# Autodesk Inventor assembly: Stator
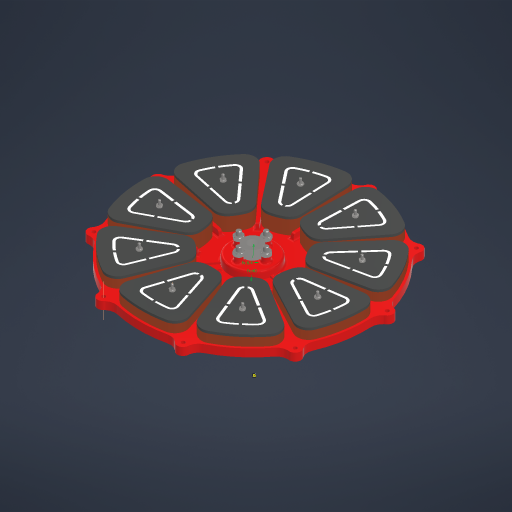
[picture p0: Inventor's stored thumbnail of the model, 512x512]
Saved by Autodesk Inventor 2023.1 (Build 271208000, 208)
## iProperties
Created: 2022-07-30
Part Number: Stator
Document SubType Name: Assembly
Designer: ABL
Author: ABL
## Documents named in this file (11)
- C:\GitHubRepos\PHYS-12-Website\content\portfolio\Final Project\CAD\Axial Flux Motor iProject\Stator.iam
- C:\GitHubRepos\PHYS-12-Website\content\portfolio\Final Project\CAD\Axial Flux Motor iProject\StatorBody.ipt
- C:\GitHubRepos\PHYS-12-Website\content\portfolio\Final Project\CAD\Axial Flux Motor iProject\CoilRing.ipt
- C:\GitHubRepos\PHYS-12-Website\content\portfolio\The Everybolt\MetricSocketBolt.ipt
- C:\GitHubRepos\PHYS-12-Website\content\portfolio\Final Project\CAD\Axial Flux Motor iProject\Fasteners\statorMountBolt.ipt
- C:\GitHubRepos\PHYS-12-Website\content\portfolio\Final Project\CAD\Axial Flux Motor iProject\Fasteners\statorMountHexNut.ipt
- C:\GitHubRepos\PHYS-12-Website\content\portfolio\The Everybolt\MetricHexNut.ipt
- C:\GitHubRepos\PHYS-12-Website\content\portfolio\Final Project\CAD\Axial Flux Motor iProject\FlangeCoupling.ipt
- C:\GitHubRepos\PHYS-12-Website\content\portfolio\Final Project\CAD\Axial Flux Motor iProject\Fasteners\statorCoilBolt.ipt
- C:\GitHubRepos\PHYS-12-Website\content\portfolio\Final Project\CAD\Axial Flux Motor iProject\Fasteners\statorCoilHexNut.ipt
- C:\GitHubRepos\PHYS-12-Website\content\portfolio\Final Project\CAD\Axial Flux Motor iProject\MotorGlobalParameters.xlsx
## Components (37 placed, 7 different names)
1. StatorBody:1 — Flush:1, Mate:1, Mate:2, Mate:3, Mate:4, Tangent:1, Mate:5, Mate:7, Mate:9, Mate:10, Mate:11
2. FlangeCoupling:1 — Mate:6, Mate:7, Mate:8, Mate:9
3. CoilRing:1 — Flush:1, Mate:1, Mate:2, Mate:12, Mate:13
4. CoilRing:2
5. CoilRing:3
6. CoilRing:4
7. CoilRing:5
8. CoilRing:6
9. CoilRing:7
10. CoilRing:8
11. CoilRing:9
12. statorCoilBolt:5 — Mate:10, Mate:11
13. statorCoilHexNut:5 — Mate:12, Mate:13
14. statorCoilBolt:6
15. statorCoilHexNut:6
16. statorCoilBolt:7
17. statorCoilHexNut:7
18. statorCoilBolt:8
19. statorCoilHexNut:8
20. statorCoilBolt:9
21. statorCoilHexNut:9
22. statorCoilBolt:10
23. statorCoilHexNut:10
24. statorCoilBolt:11
25. statorCoilHexNut:11
26. statorCoilBolt:12
27. statorCoilHexNut:12
28. statorCoilBolt:13
29. statorCoilHexNut:13
30. statorMountBolt:1 — Mate:5, Mate:8, Mate:6
31. statorMountHexNut:1 — Mate:3, Mate:4, Tangent:1
32. statorMountBolt:2
33. statorMountHexNut:2
34. statorMountBolt:3
35. statorMountHexNut:3
36. statorMountBolt:4
37. statorMountHexNut:4
## Component patterns: Coils (9 elements), (9 elements, first: statorCoilBolt:5 + statorCoilHexNut:5), (4 elements, first: statorMountBolt:1 + statorMountHexNut:1)
## Relationships (15: Mate 13, Flush 1, Tangent 1)
- Flush:1: StatorBody:1 ↔ CoilRing:1
- Mate:1: StatorBody:1 ↔ CoilRing:1
- Mate:2: StatorBody:1 ↔ CoilRing:1
- Mate:3: StatorBody:1 ↔ statorMountHexNut:1
- Mate:4: StatorBody:1 ↔ statorMountHexNut:1
- Tangent:1: StatorBody:1 ↔ statorMountHexNut:1
- Mate:5: StatorBody:1 ↔ statorMountBolt:1
- Mate:6: FlangeCoupling:1 ↔ statorMountBolt:1
- Mate:7: StatorBody:1 ↔ FlangeCoupling:1
- Mate:8: FlangeCoupling:1 ↔ statorMountBolt:1
- Mate:9: StatorBody:1 ↔ FlangeCoupling:1
- Mate:10: StatorBody:1 ↔ statorCoilBolt:5
- Mate:11: StatorBody:1 ↔ statorCoilBolt:5
- Mate:12: CoilRing:1 ↔ statorCoilHexNut:5
- Mate:13: CoilRing:1 ↔ statorCoilHexNut:5
## Named parameters: gap = 0.1 mm, airgap = 0.4 mm, wallgap = 2 mm, driveMagnet_length = 60 mm, driveMagnet_width = 10 mm, driveMagnet_height = 5 mm, driveMagnet_numStacked = 2, halbachMagnet_length = 60 mm, halbachMagnet_width = 10 mm, halbachMagnet_height = 3 mm, halbachMagnet_numStacked = 2, rotorBandBolt_diameter = 2 mm, rotorBandBolt_headDiameter = 3.98 mm, rotorBandBolt_headHeight = 2 mm, rotorBandBolt_shaftLength = 20 mm, rotorBandHexNut_sideToSide = 4 mm, rotorBandHexNut_height = 1.2 mm, rotorBandSquareNut_sideLength = 4 mm, rotorBandSquareNut_height = 1.2 mm, sensorMagnet_diameter = 5 mm, sensorMagnet_height = 2.66667 mm, numMagnetSets = 12, numElectromagnets = 9, driveMagnet_centerSpacingRadius = 38.96113 mm, rotorRadius = 101.16113 mm, rotorThickness = 14.1 mm, rotor_mountingLipHeight = 8 mm, shaftDiameter = 8 mm, flangeBearing_innerDiameter = 8 mm, flangeBearing_outerDiameter = 16 mm, flangeBearing_flangeDiameter = 18 mm, flangeBearing_height = 5 mm, flangeBearing_flangeHeight = 1 mm, statorThickness = 16 mm, rotorBandThickness = 4.1 mm, shaftLength = 200 mm, flangeCoupling_collarOuterDiameter = 16 mm, flangeCoupling_flangeHoleEdgeToEdge = 2.05 mm, flangeCoupling_innerDiameter = 8 mm, flangeCoupling_flangeHoleDiameter = 3.9 mm, flangeCoupling_flangeHeight = 3.1 mm, flangeCoupling_collarHeight = 10 mm, flangeCoupling_flangeDiameter = 32 mm, flangeCoupling_height = 13.1 mm, flangeCoupling_mountHoleDiameter = 3.9 mm, flangeCoupling_mountHoleEdgeToEdge = 2.05 mm, statorRadius = 99.16113 mm, coilThickness = 12 mm, statorMountBolt_diameter = 4 mm, statorMountBolt_headDiameter = 7 mm, statorMountBolt_headHeight = 4 mm, statorMountBolt_shaftLength = 17.1 mm, statorMountHexNut_height = 4 mm, statorMountHexNut_sideToSide = 8 mm, sensorMagnet_ringRadius = 23.48057 mm, coil_percentCoverage = 0.6, statorSpokeDegrees = 4 deg, coil_bulge = 3 mm, coil_cornerRadius = 10 mm, coil_width = 10 mm, statorCoilBolt_shaftLength = 19.3 mm, statorCoilHexNut_height = 1.2 mm, statorCoilBolt_headHeight = 2 mm, statorCoilBolt_diameter = 2 mm, statorCoilBolt_headDiameter = 3.98 mm, statorCoilHexNut_sideToSide = 4 mm, magnetWire_gauge = 20, magnetWire_outerDiameter = 0.8128 mm, printingLayerHeight = 0.2 mm, circuitBoard_height = 1.6 mm, hallEffectSensor_width = 1.6 mm, hallEffectSensor_length = 3 mm, hallEffectSensor_height = 1.1 mm, hallEffectSensor_pinLength = 0.6 mm, circuitboardMountHexNut_height = 1.2 mm, circuitboardMountHexNut_sideToSide = 4 mm, circuitboardMountBolt_headHeight = 2 mm, circuitboardMountBolt_shaftLength = 12 mm, circuitboardMountBolt_diameter = 2 mm, circuitboardMountBolt_headDiameter = 3.98 mm, statorShellBolt_headDiameter = 5.68 mm, statorShellHexNut_height = 2.3 mm, statorShellBolt_shaftLength = 12.6 mm, statorShellBolt_headHeight = 3 mm, statorShellHexNut_sideToSide = 5.3 mm, statorShellBolt_diameter = 3 mm, statorShellBolt_countersinkDepth = 3.4 mm, flangeCoupling_mountHoleCenterToCouplingCenter = 12 mm
